# Autodesk Inventor assembly: Intake Pivot Assembly
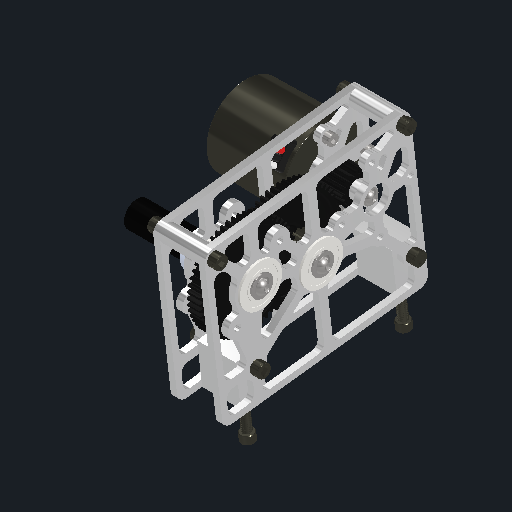
[picture p0: Inventor's stored thumbnail of the model, 512x512]
Saved by Autodesk Inventor 2024.2 (Build 282272000, 272)
## iProperties
Created: 2024-08-01
Part Number: Intake Pivot Assembly
Document SubType Name: Assembly
Designer: Kenji
Mass: 1227 g
Surface Area: 1748.77 cm^2
Volume: 303.864 cm^3
Density: 4.03801 g/cm^3
Author: Kenji
## Documents named in this file (23)
- C:\Users\bobsb\OneDrive\Documents\GitHub\1622-2024-Summer-CAD-A-Thon\Intake\Intake Pivot Assembly.iam
- C:\Users\bobsb\OneDrive\Documents\GitHub\1622-2024-Summer-CAD-A-Thon\COTS Library\Motors\COTS_REV-21-1650-V1.1_Neo1.1.ipt
- C:\Users\bobsb\OneDrive\Documents\GitHub\1622-2024-Summer-CAD-A-Thon\COTS Library\Motion\Bearings\COTS_WCP-0783_1.125ODHexBearing.ipt
- C:\Users\bobsb\OneDrive\Documents\GitHub\1622-2024-Summer-CAD-A-Thon\COTS Library\Fasteners\Bolts\Socket-Head\10-32\COTS_91251A340__3-18in long_Black-Oxide Alloy Steel Socket Head.ipt
- C:\Users\bobsb\OneDrive\Documents\GitHub\1622-2024-Summer-CAD-A-Thon\Intake\Intake Pivot Spacer 1.ipt
- C:\Users\bobsb\OneDrive\Documents\GitHub\1622-2024-Summer-CAD-A-Thon\Intake\Intake Pivot Spacer 2.ipt
- C:\Users\bobsb\OneDrive\Documents\GitHub\1622-2024-Summer-CAD-A-Thon\Intake\Intake Pivot Hex Shaft.ipt
- C:\Users\bobsb\OneDrive\Documents\GitHub\1622-2024-Summer-CAD-A-Thon\Intake\Intake Pivot Spacer 3.ipt
- C:\Users\bobsb\OneDrive\Documents\GitHub\1622-2024-Summer-CAD-A-Thon\COTS Library\Fasteners\Bolts\Socket-Head\0.25-20\COTS_91251A537_Black-Oxide Alloy Steel Socket Head Screw.ipt
- C:\Users\bobsb\OneDrive\Documents\GitHub\1622-2024-Summer-CAD-A-Thon\COTS Library\Fasteners\Washers\COTS_90107A029_316 Stainless Steel Washer.ipt
- C:\Users\bobsb\OneDrive\Documents\GitHub\1622-2024-Summer-CAD-A-Thon\COTS Library\Fasteners\Washers\COTS_91860A047_Size10Washer.ipt
- C:\Users\bobsb\OneDrive\Documents\GitHub\1622-2024-Summer-CAD-A-Thon\COTS Library\Fasteners\Bolts\Button-Head\10-32\COTS_92949A265_1-2in long Stainless Steel Button Head Screw.ipt
- C:\Users\bobsb\OneDrive\Documents\GitHub\1622-2024-Summer-CAD-A-Thon\Intake\Intake Pivot Gearbox Plate.ipt
- C:\Users\bobsb\OneDrive\Documents\GitHub\1622-2024-Summer-CAD-A-Thon\COTS Library\Motion\Gears\20DP gears\Steel\0.5in hex\COTS_WCP-0733_Steel_18T20DPGear.ipt
- C:\Users\bobsb\OneDrive\Documents\GitHub\1622-2024-Summer-CAD-A-Thon\COTS Library\Fasteners\Bolts\Button-Head\0.25-20\COTS_0.25-20_ButtonHead_0.5inlong_StainlessSteel_92949A537.ipt
- C:\Users\bobsb\OneDrive\Documents\GitHub\1622-2024-Summer-CAD-A-Thon\Intake\Intake Pivot Billet.ipt
- C:\Users\bobsb\OneDrive\Documents\GitHub\1622-2024-Summer-CAD-A-Thon\COTS Library\Fasteners\Bolts\Socket-Head\0.25-20\COTS_91251A539_Black-Oxide Alloy Steel Socket Head Screw (1).ipt
- C:\Users\bobsb\OneDrive\Documents\GitHub\1622-2024-Summer-CAD-A-Thon\COTS Library\Fasteners\Shaft Collars\COTS_WCP-0799_0.5inchHexShaftCollar.ipt
- C:\Users\bobsb\OneDrive\Documents\GitHub\1622-2024-Summer-CAD-A-Thon\Intake\Intake Pivot Spacer 4.ipt
- C:\Users\bobsb\OneDrive\Documents\GitHub\1622-2024-Summer-CAD-A-Thon\COTS Library\Fasteners\Bolts\Socket-Head\0.25-20\COTS_90044A123_Black-Oxide Alloy Steel Socket Head Screw.ipt
- C:\Users\bobsb\OneDrive\Documents\GitHub\1622-2024-Summer-CAD-A-Thon\COTS Library\Motion\Gears\Motor Gears\COTS_WCP-1236_16T20DPMotorGear.ipt
- C:\Users\bobsb\OneDrive\Documents\GitHub\1622-2024-Summer-CAD-A-Thon\COTS Library\Motion\Gears\20DP gears\Steel\0.5in hex\COTS_WCP-0185_Steel_56T20DPGear.ipt
- C:\Users\bobsb\OneDrive\Documents\GitHub\1622-2024-Summer-CAD-A-Thon\COTS Library\Motion\Gears\20DP gears\Steel\0.5in hex\COTS_WCP-0184_Steel_54T20DPGear.ipt
## Components (42 placed, 22 different names)
1. COTS_REV-21-1650-V1.1_Neo1.1:1 — Mate:33, Mate:63, Mate:75, Mate:96, Mate:97, Mate:150
2. COTS_WCP-0783_1.125ODHexBearing:1 — Flush:3, Mate:56, Mate:85, Mate:86, Flush:4, Mate:113, Mate:127, Mate:128, Mate:156
3. COTS_WCP-0783_1.125ODHexBearing:2 — Mate:81, Mate:82, Mate:98, Mate:108, Mate:133
4. COTS_WCP-0783_1.125ODHexBearing:3 — Mate:60, Mate:87, Mate:88, Flush:4, Mate:114, Mate:115, Mate:142, Mate:143, Mate:155
5. COTS_WCP-0783_1.125ODHexBearing:4 — Mate:83, Mate:84, Mate:154
6. COTS_91251A340__3-18in long_Black-Oxide Alloy Steel Socket Head:2 — Mate:100, Mate:104
7. COTS_91251A340__3-18in long_Black-Oxide Alloy Steel Socket Head:4 — Mate:99, Mate:103
8. COTS_91251A340__3-18in long_Black-Oxide Alloy Steel Socket Head:6 — Mate:101, Mate:102
9. Intake Pivot Spacer 1:1 — Mate:33, Mate:76, Mate:152
10. Intake Pivot Spacer 2:1 — Mate:113, Mate:114, Mate:115
11. Intake Pivot Hex Shaft:2 — Flush:3, Mate:59, Mate:117
12. Intake Pivot Spacer 3:2 — Mate:89, Mate:90, Mate:91, Mate:92, Mate:93
13. COTS_91251A537_Black-Oxide Alloy Steel Socket Head Screw:1 — Mate:90, Mate:94
14. COTS_91251A537_Black-Oxide Alloy Steel Socket Head Screw:2 — Mate:89, Mate:95
15. COTS_91251A537_Black-Oxide Alloy Steel Socket Head Screw:7 — Mate:57, Mate:58, Mate:59, Mate:98
16. COTS_90107A029_316 Stainless Steel Washer:1 — Mate:56, Mate:116, Mate:117, Mate:118
17. COTS_90107A029_316 Stainless Steel Washer:2 — Mate:57, Mate:58, Mate:60, Mate:153
18. COTS_91860A047_Size10Washer:1 — Mate:61, Mate:62, Mate:63, Mate:76
19. COTS_92949A265_1-2in long Stainless Steel Button Head Screw:1 — Mate:61, Mate:62
20. Intake Pivot Gearbox Plate:1 — Mate:73, Mate:74, Mate:81, Mate:82, Mate:85, Mate:86, Mate:91, Mate:92, Mate:94, Mate:120, Mate:121, Mate:124, Mate:129, Mate:130, Mate:135, Mate:137, Mate:138, Mate:141
21. Intake Pivot Gearbox Plate:2 — Mate:73, Mate:74, Mate:75, Mate:83, Mate:84, Mate:87, Mate:88, Mate:93, Mate:95, Mate:96, Mate:97, Mate:99, Mate:100, Mate:101, Mate:102, Mate:103, Mate:104, Mate:105, Mate:106, Mate:119, Mate:122, Mate:123, Mate:131, Mate:132, Flush:5, Flush:6, Mate:134, Mate:136, Mate:139, Mate:140, Mate:151
22. COTS_91251A340__3-18in long_Black-Oxide Alloy Steel Socket Head:7 — Mate:105, Mate:106
23. COTS_WCP-0733_Steel_18T20DPGear:1 — Mate:108, Mate:133
24. COTS_0.25-20_ButtonHead_0.5inlong_StainlessSteel_92949A537:1 — Mate:116, Mate:118
25. Intake Pivot Spacer 3:3 — Mate:119, Mate:120
26. COTS_91251A537_Black-Oxide Alloy Steel Socket Head Screw:8 — Mate:121, Mate:124
27. COTS_91251A537_Black-Oxide Alloy Steel Socket Head Screw:9 — Mate:122, Mate:123
28. COTS_0.25-20_ButtonHead_0.5inlong_StainlessSteel_92949A537:2 — Mate:125, Mate:126
29. COTS_90107A029_316 Stainless Steel Washer:4 — Mate:125, Mate:126, Mate:127, Mate:128
30. Intake Pivot Billet:1 — Mate:129, Mate:132, Flush:5, Mate:147, Mate:149
31. Intake Pivot Billet:2 — Mate:130, Mate:131, Flush:6, Mate:146, Mate:148
32. COTS_91251A539_Black-Oxide Alloy Steel Socket Head Screw (1):1 — Mate:134, Mate:136
33. COTS_91251A539_Black-Oxide Alloy Steel Socket Head Screw (1):2 — Mate:135, Mate:137
34. COTS_91251A539_Black-Oxide Alloy Steel Socket Head Screw (1):3 — Mate:138, Mate:141
35. COTS_91251A539_Black-Oxide Alloy Steel Socket Head Screw (1):4 — Mate:139, Mate:140
36. COTS_WCP-0799_0.5inchHexShaftCollar:1 — Mate:142, Mate:143, Mate:144, Mate:145
37. Intake Pivot Spacer 4:1 — Mate:144, Mate:145
38. COTS_90044A123_Black-Oxide Alloy Steel Socket Head Screw:1 — Mate:147, Mate:149
39. COTS_90044A123_Black-Oxide Alloy Steel Socket Head Screw:2 — Mate:146, Mate:148
40. COTS_WCP-1236_16T20DPMotorGear:1 — Mate:150, Mate:151, Mate:152
41. COTS_WCP-0185_Steel_56T20DPGear:1 — Mate:153, Mate:154
42. COTS_WCP-0184_Steel_54T20DPGear:1 — Mate:155, Mate:156
## Relationships (88: Mate 84, Flush 4)
- Mate:33: COTS_REV-21-1650-V1.1_Neo1.1:1 ↔ Intake Pivot Spacer 1:1
- Flush:3: COTS_WCP-0783_1.125ODHexBearing:1 ↔ Intake Pivot Hex Shaft:2
- Mate:56: COTS_WCP-0783_1.125ODHexBearing:1 ↔ COTS_90107A029_316 Stainless Steel Washer:1
- Mate:57: COTS_91251A537_Black-Oxide Alloy Steel Socket Head Screw:7 ↔ COTS_90107A029_316 Stainless Steel Washer:2
- Mate:58: COTS_91251A537_Black-Oxide Alloy Steel Socket Head Screw:7 ↔ COTS_90107A029_316 Stainless Steel Washer:2
- Mate:59: Intake Pivot Hex Shaft:2 ↔ COTS_91251A537_Black-Oxide Alloy Steel Socket Head Screw:7
- Mate:60: COTS_WCP-0783_1.125ODHexBearing:3 ↔ COTS_90107A029_316 Stainless Steel Washer:2
- Mate:61: COTS_91860A047_Size10Washer:1 ↔ COTS_92949A265_1-2in long Stainless Steel Button Head Screw:1
- Mate:62: COTS_91860A047_Size10Washer:1 ↔ COTS_92949A265_1-2in long Stainless Steel Button Head Screw:1
- Mate:63: COTS_REV-21-1650-V1.1_Neo1.1:1 ↔ COTS_91860A047_Size10Washer:1
- Mate:73: Intake Pivot Gearbox Plate:1 ↔ Intake Pivot Gearbox Plate:2
- Mate:74: Intake Pivot Gearbox Plate:1 ↔ Intake Pivot Gearbox Plate:2
- Mate:75: COTS_REV-21-1650-V1.1_Neo1.1:1 ↔ Intake Pivot Gearbox Plate:2
- Mate:76: Intake Pivot Spacer 1:1 ↔ COTS_91860A047_Size10Washer:1
- Mate:81: COTS_WCP-0783_1.125ODHexBearing:2 ↔ Intake Pivot Gearbox Plate:1
- Mate:82: COTS_WCP-0783_1.125ODHexBearing:2 ↔ Intake Pivot Gearbox Plate:1
- Mate:83: COTS_WCP-0783_1.125ODHexBearing:4 ↔ Intake Pivot Gearbox Plate:2
- Mate:84: COTS_WCP-0783_1.125ODHexBearing:4 ↔ Intake Pivot Gearbox Plate:2
- Mate:85: COTS_WCP-0783_1.125ODHexBearing:1 ↔ Intake Pivot Gearbox Plate:1
- Mate:86: COTS_WCP-0783_1.125ODHexBearing:1 ↔ Intake Pivot Gearbox Plate:1
- Mate:87: COTS_WCP-0783_1.125ODHexBearing:3 ↔ Intake Pivot Gearbox Plate:2
- Mate:88: COTS_WCP-0783_1.125ODHexBearing:3 ↔ Intake Pivot Gearbox Plate:2
- Mate:89: Intake Pivot Spacer 3:2 ↔ COTS_91251A537_Black-Oxide Alloy Steel Socket Head Screw:2
- Mate:90: Intake Pivot Spacer 3:2 ↔ COTS_91251A537_Black-Oxide Alloy Steel Socket Head Screw:1
- Mate:91: Intake Pivot Spacer 3:2 ↔ Intake Pivot Gearbox Plate:1
- Mate:92: Intake Pivot Spacer 3:2 ↔ Intake Pivot Gearbox Plate:1
- Mate:93: Intake Pivot Spacer 3:2 ↔ Intake Pivot Gearbox Plate:2
- Mate:94: COTS_91251A537_Black-Oxide Alloy Steel Socket Head Screw:1 ↔ Intake Pivot Gearbox Plate:1
- Mate:95: COTS_91251A537_Black-Oxide Alloy Steel Socket Head Screw:2 ↔ Intake Pivot Gearbox Plate:2
- Mate:96: COTS_REV-21-1650-V1.1_Neo1.1:1 ↔ Intake Pivot Gearbox Plate:2
- Mate:97: COTS_REV-21-1650-V1.1_Neo1.1:1 ↔ Intake Pivot Gearbox Plate:2
- Mate:98: COTS_WCP-0783_1.125ODHexBearing:2 ↔ COTS_91251A537_Black-Oxide Alloy Steel Socket Head Screw:7
- Mate:99: COTS_91251A340__3-18in long_Black-Oxide Alloy Steel Socket Head:4 ↔ Intake Pivot Gearbox Plate:2
- Mate:100: COTS_91251A340__3-18in long_Black-Oxide Alloy Steel Socket Head:2 ↔ Intake Pivot Gearbox Plate:2
- Mate:101: COTS_91251A340__3-18in long_Black-Oxide Alloy Steel Socket Head:6 ↔ Intake Pivot Gearbox Plate:2
- Mate:102: COTS_91251A340__3-18in long_Black-Oxide Alloy Steel Socket Head:6 ↔ Intake Pivot Gearbox Plate:2
- Mate:103: COTS_91251A340__3-18in long_Black-Oxide Alloy Steel Socket Head:4 ↔ Intake Pivot Gearbox Plate:2
- Mate:104: COTS_91251A340__3-18in long_Black-Oxide Alloy Steel Socket Head:2 ↔ Intake Pivot Gearbox Plate:2
- Mate:105: Intake Pivot Gearbox Plate:2 ↔ COTS_91251A340__3-18in long_Black-Oxide Alloy Steel Socket Head:7
- Mate:106: Intake Pivot Gearbox Plate:2 ↔ COTS_91251A340__3-18in long_Black-Oxide Alloy Steel Socket Head:7
- Mate:108: COTS_WCP-0783_1.125ODHexBearing:2 ↔ COTS_WCP-0733_Steel_18T20DPGear:1
- Flush:4: COTS_WCP-0783_1.125ODHexBearing:1 ↔ COTS_WCP-0783_1.125ODHexBearing:3
- Mate:113: COTS_WCP-0783_1.125ODHexBearing:1 ↔ Intake Pivot Spacer 2:1
- Mate:114: COTS_WCP-0783_1.125ODHexBearing:3 ↔ Intake Pivot Spacer 2:1
- Mate:115: COTS_WCP-0783_1.125ODHexBearing:3 ↔ Intake Pivot Spacer 2:1
- Mate:116: COTS_90107A029_316 Stainless Steel Washer:1 ↔ COTS_0.25-20_ButtonHead_0.5inlong_StainlessSteel_92949A537:1
- Mate:117: Intake Pivot Hex Shaft:2 ↔ COTS_90107A029_316 Stainless Steel Washer:1
- Mate:118: COTS_90107A029_316 Stainless Steel Washer:1 ↔ COTS_0.25-20_ButtonHead_0.5inlong_StainlessSteel_92949A537:1
- Mate:119: Intake Pivot Gearbox Plate:2 ↔ Intake Pivot Spacer 3:3
- Mate:120: Intake Pivot Gearbox Plate:1 ↔ Intake Pivot Spacer 3:3
- Mate:121: Intake Pivot Gearbox Plate:1 ↔ COTS_91251A537_Black-Oxide Alloy Steel Socket Head Screw:8
- Mate:122: Intake Pivot Gearbox Plate:2 ↔ COTS_91251A537_Black-Oxide Alloy Steel Socket Head Screw:9
- Mate:123: Intake Pivot Gearbox Plate:2 ↔ COTS_91251A537_Black-Oxide Alloy Steel Socket Head Screw:9
- Mate:124: Intake Pivot Gearbox Plate:1 ↔ COTS_91251A537_Black-Oxide Alloy Steel Socket Head Screw:8
- Mate:125: COTS_0.25-20_ButtonHead_0.5inlong_StainlessSteel_92949A537:2 ↔ COTS_90107A029_316 Stainless Steel Washer:4
- Mate:126: COTS_0.25-20_ButtonHead_0.5inlong_StainlessSteel_92949A537:2 ↔ COTS_90107A029_316 Stainless Steel Washer:4
- Mate:127: COTS_WCP-0783_1.125ODHexBearing:1 ↔ COTS_90107A029_316 Stainless Steel Washer:4
- Mate:128: COTS_WCP-0783_1.125ODHexBearing:1 ↔ COTS_90107A029_316 Stainless Steel Washer:4
- Mate:129: Intake Pivot Gearbox Plate:1 ↔ Intake Pivot Billet:1
- Mate:130: Intake Pivot Gearbox Plate:1 ↔ Intake Pivot Billet:2
- Mate:131: Intake Pivot Gearbox Plate:2 ↔ Intake Pivot Billet:2
- Mate:132: Intake Pivot Gearbox Plate:2 ↔ Intake Pivot Billet:1
- Flush:5: Intake Pivot Gearbox Plate:2 ↔ Intake Pivot Billet:1
- Flush:6: Intake Pivot Gearbox Plate:2 ↔ Intake Pivot Billet:2
- Mate:133: COTS_WCP-0783_1.125ODHexBearing:2 ↔ COTS_WCP-0733_Steel_18T20DPGear:1
- Mate:134: Intake Pivot Gearbox Plate:2 ↔ COTS_91251A539_Black-Oxide Alloy Steel Socket Head Screw (1):1
- Mate:135: Intake Pivot Gearbox Plate:1 ↔ COTS_91251A539_Black-Oxide Alloy Steel Socket Head Screw (1):2
- Mate:136: Intake Pivot Gearbox Plate:2 ↔ COTS_91251A539_Black-Oxide Alloy Steel Socket Head Screw (1):1
- Mate:137: Intake Pivot Gearbox Plate:1 ↔ COTS_91251A539_Black-Oxide Alloy Steel Socket Head Screw (1):2
- Mate:138: Intake Pivot Gearbox Plate:1 ↔ COTS_91251A539_Black-Oxide Alloy Steel Socket Head Screw (1):3
- Mate:139: Intake Pivot Gearbox Plate:2 ↔ COTS_91251A539_Black-Oxide Alloy Steel Socket Head Screw (1):4
- Mate:140: Intake Pivot Gearbox Plate:2 ↔ COTS_91251A539_Black-Oxide Alloy Steel Socket Head Screw (1):4
- Mate:141: Intake Pivot Gearbox Plate:1 ↔ COTS_91251A539_Black-Oxide Alloy Steel Socket Head Screw (1):3
- Mate:142: COTS_WCP-0783_1.125ODHexBearing:3 ↔ COTS_WCP-0799_0.5inchHexShaftCollar:1
- Mate:143: COTS_WCP-0783_1.125ODHexBearing:3 ↔ COTS_WCP-0799_0.5inchHexShaftCollar:1
- Mate:144: COTS_WCP-0799_0.5inchHexShaftCollar:1 ↔ Intake Pivot Spacer 4:1
- Mate:145: COTS_WCP-0799_0.5inchHexShaftCollar:1 ↔ Intake Pivot Spacer 4:1
- Mate:146: Intake Pivot Billet:2 ↔ COTS_90044A123_Black-Oxide Alloy Steel Socket Head Screw:2
- Mate:147: Intake Pivot Billet:1 ↔ COTS_90044A123_Black-Oxide Alloy Steel Socket Head Screw:1
- Mate:148 (25.4 mm): Intake Pivot Billet:2 ↔ COTS_90044A123_Black-Oxide Alloy Steel Socket Head Screw:2
- Mate:149 (25.4 mm): Intake Pivot Billet:1 ↔ COTS_90044A123_Black-Oxide Alloy Steel Socket Head Screw:1
- Mate:150: COTS_REV-21-1650-V1.1_Neo1.1:1 ↔ COTS_WCP-1236_16T20DPMotorGear:1
- Mate:151: Intake Pivot Gearbox Plate:2 ↔ COTS_WCP-1236_16T20DPMotorGear:1
- Mate:152: Intake Pivot Spacer 1:1 ↔ COTS_WCP-1236_16T20DPMotorGear:1
- Mate:153: COTS_90107A029_316 Stainless Steel Washer:2 ↔ COTS_WCP-0185_Steel_56T20DPGear:1
- Mate:154: COTS_WCP-0783_1.125ODHexBearing:4 ↔ COTS_WCP-0185_Steel_56T20DPGear:1
- Mate:155: COTS_WCP-0783_1.125ODHexBearing:3 ↔ COTS_WCP-0184_Steel_54T20DPGear:1
- Mate:156: COTS_WCP-0783_1.125ODHexBearing:1 ↔ COTS_WCP-0184_Steel_54T20DPGear:1
